# Autodesk Inventor assembly: FE-00029
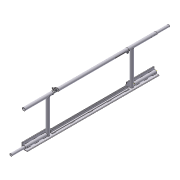
[picture p0: Inventor's stored thumbnail of the model, 180x180]
Saved by Autodesk Inventor 2012 (Build 160160000, 160)
## iProperties
Created: 2009-01-02
Part Number: FE-00029
Document SubType Name: Assembly
Designer: dfoster
Author: dfoster
## Documents named in this file (12)
- C:\Data Folder\FRC 2012 Field\Components\FE-00029.iam
- C:\Data Folder\FRC 2012 Field\Components\FE-00006.iam
- C:\Data Folder\FRC 2012 Field\Components\FE-00027.ipt
- C:\Data Folder\FRC 2012 Field\Components\FE-00026.ipt
- C:\Data Folder\FRC 2012 Field\Components\FE-00028.ipt
- C:\Data Folder\FRC 2012 Field\Components\FE-00031.ipt
- C:\Data Folder\FRC 2012 Field\Components\HW-00010.ipt
- C:\Data Folder\FRC 2012 Field\Components\ASTM F436 - 1_2(1).ipt
- C:\Data Folder\FRC 2012 Field\Components\ANSI B18.3 - 3_8-16 UNC - 2.125(18).ipt
- C:\Data Folder\FRC 2012 Field\Components\HW-00026.ipt
- C:\Data Folder\FRC 2012 Field\Components\ANSI B18.3 - 1_4-20 UNC - UNC - 0.75(1).ipt
- C:\Data Folder\FRC 2012 Field\Components\PP-00012.ipt
## Components (19 placed, 11 different names)
1. FE-00006:1 [sub-assembly] — Mate:5, Tangent:1, Mate:7, Mate:8, Tangent:3, Tangent:5, Mate:19, Mate:20, Tangent:7, Tangent:8, Mate:24, Mate:25, Mate:26, Mate:27, Mate:28, Mate:29
2. FE-00027:1 — Mate:5, Tangent:1, Mate:6, Mate:15, Mate:16
3. FE-00027:2 — Mate:6, Tangent:2, Angle:1, Insert:1, Mate:21, Mate:22
4. FE-00026:1 — Mate:24, Mate:25
5. FE-00026:2 — Mate:26, Mate:27
6. FE-00028:1 — Mate:7, Mate:8, Tangent:2, Angle:1, Mate:9, Mate:10, Tangent:9, Tangent:10, Tangent:11
7. FE-00031:1 — Mate:9, Mate:10, Mate:23
8. Circular Washer (Inch) 1/2:1 — Insert:1
9. Hexagon Socket Head Shoulder Screw - Inch 0.500 x 1.5 ANSI B18.3:1 — Mate:15, Mate:16, Mate:17, Mate:18
10. HW-00026:1 — Mate:17, Mate:18
11. Hexagon Socket Button Head Cap Screw - Inch 1/4 - 20 x 3/4:1 — Mate:20, Tangent:8
12. Hexagon Socket Button Head Cap Screw - Inch 1/4 - 20 x 3/4:2 — Mate:19, Tangent:7
13. Hexagon Socket Button Head Cap Screw - Inch 1/4 - 20 x 3/4:3 — Mate:22, Tangent:10
14. Hexagon Socket Button Head Cap Screw - Inch 1/4 - 20 x 3/4:4 — Mate:21, Tangent:9
15. PP-00012:1 — Mate:23, Tangent:11
16. HW-00010:1 — Tangent:5, Mate:28
17. HW-00010:5
18. HW-00010:4 — Tangent:3, Mate:29
19. HW-00010:6
## Component patterns: (2 elements, first: HW-00010:1), (2 elements, first: HW-00010:4)
## Relationships (32: Mate 21, Tangent 9, Angle 1, Insert 1)
- Mate:5: FE-00006:1 ↔ FE-00027:1
- Tangent:1: FE-00006:1 ↔ FE-00027:1
- Mate:6: FE-00027:1 ↔ FE-00027:2
- Mate:7: FE-00006:1 ↔ FE-00028:1
- Mate:8 (1.27 mm): FE-00006:1 ↔ FE-00028:1
- Tangent:2: FE-00027:2 ↔ FE-00028:1
- Angle:1 (-90 deg): FE-00027:2 ↔ FE-00028:1
- Mate:9: FE-00028:1 ↔ FE-00031:1
- Mate:10: FE-00028:1 ↔ FE-00031:1
- Tangent:3: FE-00006:1 ↔ HW-00010:4
- Tangent:5: FE-00006:1 ↔ HW-00010:1
- Insert:1: FE-00027:2 ↔ Circular Washer (Inch) 1/2:1
- Mate:15: FE-00027:1 ↔ Hexagon Socket Head Shoulder Screw - Inch 0.500 x 1.5 ANSI B18.3:1
- Mate:16: FE-00027:1 ↔ Hexagon Socket Head Shoulder Screw - Inch 0.500 x 1.5 ANSI B18.3:1
- Mate:17: Hexagon Socket Head Shoulder Screw - Inch 0.500 x 1.5 ANSI B18.3:1 ↔ HW-00026:1
- Mate:18: Hexagon Socket Head Shoulder Screw - Inch 0.500 x 1.5 ANSI B18.3:1 ↔ HW-00026:1
- Mate:19: FE-00006:1 ↔ Hexagon Socket Button Head Cap Screw - Inch 1/4 - 20 x 3/4:2
- Mate:20: FE-00006:1 ↔ Hexagon Socket Button Head Cap Screw - Inch 1/4 - 20 x 3/4:1
- Tangent:7: FE-00006:1 ↔ Hexagon Socket Button Head Cap Screw - Inch 1/4 - 20 x 3/4:2
- Tangent:8: FE-00006:1 ↔ Hexagon Socket Button Head Cap Screw - Inch 1/4 - 20 x 3/4:1
- Mate:21: FE-00027:2 ↔ Hexagon Socket Button Head Cap Screw - Inch 1/4 - 20 x 3/4:4
- Mate:22: FE-00027:2 ↔ Hexagon Socket Button Head Cap Screw - Inch 1/4 - 20 x 3/4:3
- Tangent:9: FE-00028:1 ↔ Hexagon Socket Button Head Cap Screw - Inch 1/4 - 20 x 3/4:4
- Tangent:10: FE-00028:1 ↔ Hexagon Socket Button Head Cap Screw - Inch 1/4 - 20 x 3/4:3
- Mate:23: FE-00031:1 ↔ PP-00012:1
- Tangent:11 (1.27 mm): FE-00028:1 ↔ PP-00012:1
- Mate:24: FE-00006:1 ↔ FE-00026:1
- Mate:25: FE-00006:1 ↔ FE-00026:1
- Mate:26: FE-00006:1 ↔ FE-00026:2
- Mate:27: FE-00006:1 ↔ FE-00026:2
- Mate:28: FE-00006:1 ↔ HW-00010:1
- Mate:29: FE-00006:1 ↔ HW-00010:4
